# Autodesk Inventor assembly: arm
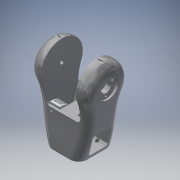
[picture p0: Inventor's stored thumbnail of the model, 180x180]
Saved by Autodesk Inventor 2019 (Build 230136000, 136)
## iProperties
Created: 2020-03-22
Part Number: arm
Document SubType Name: Assembly
Designer: james
Author: james
## Documents named in this file (5)
- F:\JimsRobot\FIRSTRobots\Design\RBX1-REMIX\arm\arm.iam
- F:\JimsRobot\FIRSTRobots\Design\RBX1-REMIX\arm\arm_body_qty1.ipt
- F:\JimsRobot\FIRSTRobots\Design\RBX1-REMIX\arm\armTens.iam
- F:\JimsRobot\FIRSTRobots\Design\Library\McMaster\StepperMotor\Nema 17 6627T670_POSITION-CONTROL DC MOTOR.ipt
- F:\JimsRobot\FIRSTRobots\Design\Library\McMaster\StepperMotor\Nema 14 6627T380_POSITION-CONTROL DC MOTOR.ipt
## Components (4 placed, 4 different names)
1. arm_body_qty1:1 — Mate:1, Mate:2, Mate:3, Mate:4
2. armTens:1 [sub-assembly] — Mate:1, Mate:2
3. Nema 17 6627T670_POSITION-CONTROL DC MOTOR:1 — Mate:4
4. Nema 14 6627T380_POSITION-CONTROL DC MOTOR:1 — Mate:3
## Relationships (4: Mate 4)
- Mate:1: arm_body_qty1:1 ↔ armTens:1
- Mate:2: arm_body_qty1:1 ↔ armTens:1
- Mate:3: arm_body_qty1:1 ↔ Nema 14 6627T380_POSITION-CONTROL DC MOTOR:1
- Mate:4: arm_body_qty1:1 ↔ Nema 17 6627T670_POSITION-CONTROL DC MOTOR:1
